# Autodesk Inventor assembly: Shapeoko_v1i
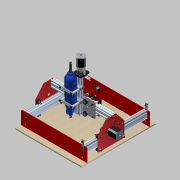
[picture p0: Inventor's stored thumbnail of the model, 180x180]
Saved by Autodesk Inventor 2012 SP1 (Build 160190100, 190)
## iProperties
Created: 2012-05-03
Part Number: Shapeoko_v1i
Document SubType Name: Assembly
Designer: ERF
Mass: 7145.43 g
Surface Area: 14170.5 cm^2
Volume: 2806.1 cm^3
Density: 2.54639 g/cm^3
Author: ERF
Title: Shapeoko v1i
## Documents named in this file (6)
- C:\Users\eford\Documents\Projects\Shapoko_v1i\Workspaces\Workspace\Projects\USER FOLDER\Edward\Shapeoko_v1i\Shapeoko_v1i.iam
- C:\Users\eford\Documents\Projects\Shapoko_v1i\Workspaces\Workspace\Projects\USER FOLDER\Edward\Shapeoko_v1i\Assemblies\SM-GA01.iam
- C:\Users\eford\Documents\Projects\Shapoko_v1i\Workspaces\Workspace\Projects\USER FOLDER\Edward\Shapeoko_v1i\Assemblies\SM-FA01.iam
- C:\Users\eford\Documents\Projects\Shapoko_v1i\Workspaces\Workspace\Projects\USER FOLDER\Edward\Shapeoko_v1i\Assemblies\SM-ZA02.iam
- C:\Users\eford\Documents\Projects\Shapoko_v1i\Workspaces\Workspace\Projects\USER FOLDER\Edward\Shapeoko_v1i\Assemblies\SM-ZA03.iam
- C:\Users\eford\Documents\Projects\Shapoko_v1i\Workspaces\Workspace\Projects\USER FOLDER\Edward\Shapeoko_v1i\Parts\SM-SWB.ipt
## Components (5 placed, 5 different names)
1. SM-GA01:1 [sub-assembly] — Mate:1, Flush:1, Mate:2, Angle:1
2. SM-FA01:1 [sub-assembly] — Mate:1, Flush:1, Mate:4, Flush:4, Flush:5
3. SM-ZA02:1 [sub-assembly] — Mate:2, Angle:1, Mate:3, Angle:2, Flush:2, Flush:3
4. SM-ZA03:1 [sub-assembly] — Mate:3, Angle:2, Flush:2, Flush:3
5. SM-SWB:1 — Mate:4, Flush:4, Flush:5
## Relationships (11: Flush 5, Mate 4, Angle 2)
- Mate:1 (6.35 mm): SM-GA01:1 ↔ SM-FA01:1
- Flush:1 (-25 mm): SM-GA01:1 ↔ SM-FA01:1
- Mate:2: SM-GA01:1 ↔ SM-ZA02:1
- Angle:1 (0 deg): SM-GA01:1 ↔ SM-ZA02:1
- Mate:3: SM-ZA02:1 ↔ SM-ZA03:1
- Angle:2 (0 deg): SM-ZA02:1 ↔ SM-ZA03:1
- Flush:2 (-20 mm): SM-ZA02:1 ↔ SM-ZA03:1
- Flush:3 (15.875 mm): SM-ZA02:1 ↔ SM-ZA03:1
- Mate:4: SM-FA01:1 ↔ SM-SWB:1
- Flush:4: SM-FA01:1 ↔ SM-SWB:1
- Flush:5 (-34.0837 mm): SM-FA01:1 ↔ SM-SWB:1
